# Autodesk Inventor assembly: Ares 2_0
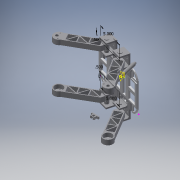
[picture p0: Inventor's stored thumbnail of the model, 180x180]
Saved by Autodesk Inventor 2018.2 (Build 222227000, 227)
## iProperties
Created: 2018-03-23
Part Number: Ares 2_0
Document SubType Name: Assembly
Designer: MIABo
Author: MIABo
## Documents named in this file (11)
- C:\Users\MIABo\OneDrive\Documents\GitHub\Ares\3D Model Files\Ares 2_0.iam
- C:\Users\MIABo\OneDrive\Documents\GitHub\Ares\3D Model Files\Frame 2.1.ipt
- C:\Users\MIABo\OneDrive\Documents\GitHub\Ares\3D Model Files\leg 3.0.ipt
- C:\Users\MIABo\OneDrive\Documents\GitHub\Ares\3D Model Files\Suspension Frame 3.0.ipt
- C:\Users\MIABo\OneDrive\Documents\GitHub\Ares\3D Model Files\Frame mount rivet.ipt
- C:\Users\MIABo\OneDrive\Documents\GitHub\Ares\3D Model Files\Leg Mount Rivet.ipt
- C:\Users\MIABo\OneDrive\Documents\GitHub\Ares\3D Model Files\Leg Spacer.ipt
- C:\Users\MIABo\OneDrive\Documents\GitHub\Ares\3D Model Files\Ultrasonic MoUnt.ipt
- C:\Users\MIABo\OneDrive\Documents\GitHub\Ares\3D Model Files\MockShock.ipt
- C:\Users\MIABo\OneDrive\Documents\GitHub\Ares\3D Model Files\LowerSpringMountFront.ipt
- C:\Users\MIABo\OneDrive\Documents\GitHub\Ares\3D Model Files\LowerSpringMountRearBracket.ipt
## Components (33 placed, 10 different names)
1. Frame 2.1:1 — Mate:1, Mate:2, Mate:3, Mate:4, Mate:5, Mate:6, Mate:8, Mate:9, Mate:10, Mate:11, Mate:13, Mate:14, Flush:1
2. leg 3.0:1 — Insert:17, Insert:18
3. leg 3.0:2 — Insert:19
4. leg 3.0:3 — Insert:24, Mate:15, Mate:16
5. leg 3.0:4 — Insert:23, Angle:1
6. Suspension Frame 3.0:1 — Mate:1, Mate:2, Mate:4, Insert:5, Insert:6, Insert:9, Insert:16, Insert:22
7. Suspension Frame 3.0:2 — Mate:3, Mate:5, Mate:6, Insert:7, Insert:8, Insert:10, Insert:15, Insert:21, Angle:1
8. Suspension Frame 3.0:3 — Mate:8, Mate:9, Mate:10, Mate:12, Insert:2, Insert:3, Insert:11, Insert:13, Insert:20
9. Suspension Frame 3.0:4 — Mate:11, Mate:12, Mate:13, Insert:1, Insert:4, Insert:12, Insert:14
10. Frame mount rivet:1 — Insert:8
11. Frame mount rivet:2 — Insert:7
12. Frame mount rivet:3 — Insert:6
13. Frame mount rivet:4 — Insert:2
14. Frame mount rivet:5 — Insert:3
15. Frame mount rivet:6 — Insert:4
16. Frame mount rivet:7 — Insert:5
17. Frame mount rivet:8 — Insert:1
18. Leg Mount Rivet:1 — Insert:9
19. Leg Mount Rivet:2 — Insert:10
20. Leg Mount Rivet:3 — Insert:11
21. Leg Mount Rivet:4 — Insert:12
22. Leg Spacer:1 — Insert:22, Insert:24
23. Leg Spacer:2 — Insert:21, Insert:23
24. Leg Spacer:3 — Insert:20
25. Leg Spacer:4 — Insert:13, Insert:19
26. Leg Spacer:5 — Insert:14, Insert:17
27. Leg Spacer:6 — Insert:15
28. Leg Spacer:7 — Insert:16
29. Leg Spacer:8 — Insert:18
30. Ultrasonic MoUnt:1 — Mate:14, Flush:1
31. MockShock:1
32. LowerSpringMountFront:1
33. LowerSpringMountRearBracket:1 — Mate:15, Mate:16
## Relationships (41: Insert 24, Mate 15, Angle 1, Flush 1)
- Mate:1: Frame 2.1:1 ↔ Suspension Frame 3.0:1
- Mate:2: Frame 2.1:1 ↔ Suspension Frame 3.0:1
- Mate:3: Frame 2.1:1 ↔ Suspension Frame 3.0:2
- Mate:4: Frame 2.1:1 ↔ Suspension Frame 3.0:1
- Mate:5: Frame 2.1:1 ↔ Suspension Frame 3.0:2
- Mate:6: Frame 2.1:1 ↔ Suspension Frame 3.0:2
- Mate:8: Frame 2.1:1 ↔ Suspension Frame 3.0:3
- Mate:9: Frame 2.1:1 ↔ Suspension Frame 3.0:3
- Mate:10: Frame 2.1:1 ↔ Suspension Frame 3.0:3
- Mate:11: Frame 2.1:1 ↔ Suspension Frame 3.0:4
- Mate:12: Suspension Frame 3.0:3 ↔ Suspension Frame 3.0:4
- Mate:13: Frame 2.1:1 ↔ Suspension Frame 3.0:4
- Insert:1 (-15.24 mm): Suspension Frame 3.0:4 ↔ Frame mount rivet:8
- Insert:2 (-15.24 mm): Suspension Frame 3.0:3 ↔ Frame mount rivet:4
- Insert:3 (-15.24 mm): Suspension Frame 3.0:3 ↔ Frame mount rivet:5
- Insert:4 (-15.24 mm): Suspension Frame 3.0:4 ↔ Frame mount rivet:6
- Insert:5 (-15.24 mm): Suspension Frame 3.0:1 ↔ Frame mount rivet:7
- Insert:6 (-15.24 mm): Suspension Frame 3.0:1 ↔ Frame mount rivet:3
- Insert:7 (-15.24 mm): Suspension Frame 3.0:2 ↔ Frame mount rivet:2
- Insert:8 (-15.24 mm): Suspension Frame 3.0:2 ↔ Frame mount rivet:1
- Insert:9: Suspension Frame 3.0:1 ↔ Leg Mount Rivet:1
- Insert:10: Suspension Frame 3.0:2 ↔ Leg Mount Rivet:2
- Insert:11: Suspension Frame 3.0:3 ↔ Leg Mount Rivet:3
- Insert:12: Suspension Frame 3.0:4 ↔ Leg Mount Rivet:4
- Insert:13: Suspension Frame 3.0:3 ↔ Leg Spacer:4
- Insert:14: Suspension Frame 3.0:4 ↔ Leg Spacer:5
- Insert:15: Suspension Frame 3.0:2 ↔ Leg Spacer:6
- Insert:16: Suspension Frame 3.0:1 ↔ Leg Spacer:7
- Insert:17: leg 3.0:1 ↔ Leg Spacer:5
- Insert:18: leg 3.0:1 ↔ Leg Spacer:8
- Insert:19: leg 3.0:2 ↔ Leg Spacer:4
- Insert:20: Suspension Frame 3.0:3 ↔ Leg Spacer:3
- Insert:21: Suspension Frame 3.0:2 ↔ Leg Spacer:2
- Insert:22: Suspension Frame 3.0:1 ↔ Leg Spacer:1
- Insert:23: leg 3.0:4 ↔ Leg Spacer:2
- Insert:24: leg 3.0:3 ↔ Leg Spacer:1
- Angle:1 (45 deg): leg 3.0:4 ↔ Suspension Frame 3.0:2
- Mate:14: Frame 2.1:1 ↔ Ultrasonic MoUnt:1
- Flush:1: Frame 2.1:1 ↔ Ultrasonic MoUnt:1
- Mate:15: leg 3.0:3 ↔ LowerSpringMountRearBracket:1
- Mate:16: leg 3.0:3 ↔ LowerSpringMountRearBracket:1
